# Autodesk Inventor assembly: MotorBlockModelisme
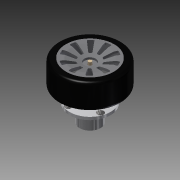
[picture p0: Inventor's stored thumbnail of the model, 180x180]
Saved by Autodesk Inventor 2014 SP1 (Build 180222100, 222)
## iProperties
Created: 2015-04-18
Part Number: MotorBlockModelisme
Document SubType Name: Assembly
Designer: david
Author: david
## Documents named in this file (5)
- C:\Users\asus\Documents\Autodesk\Projects\AUSBEEDone\Components\Motors\MotorBlockModelling.iam
- C:\Users\asus\Documents\Autodesk\Projects\AUSBEEDone\Components\Motors\Motor.iam
- C:\Users\asus\Documents\Autodesk\Projects\AUSBEEDone\Components\Modelling\Hub_Hex_12mm.ipt
- C:\Users\asus\Documents\Autodesk\Projects\AUSBEEDone\Components\Fasteners\Screw_CountersunkHead_3x10.ipt
- C:\Users\asus\Documents\Autodesk\Projects\AUSBEEDone\Components\Modelling\ModellingWheel_65mm.ipt
## Components (5 placed, 4 different names)
1. Motor:1 [sub-assembly] — Mate:1, Mate:2, Mate:5, Mate:6
2. ModellingWheel_65mm:1 — Mate:7, Angle:1, Mate:8
3. Hub_Hex_12mm:1 — Mate:1, Mate:2, Mate:3, Mate:4, Mate:7, Angle:1, Mate:8
4. Screw_CountersunkHead_3x10:1 — Mate:4, Mate:6
5. Screw_CountersunkHead_3x10:2 — Mate:3, Mate:5
## Relationships (9: Mate 8, Angle 1)
- Mate:1: Motor:1 ↔ Hub_Hex_12mm:1
- Mate:2: Motor:1 ↔ Hub_Hex_12mm:1
- Mate:3: Hub_Hex_12mm:1 ↔ Screw_CountersunkHead_3x10:2
- Mate:4: Hub_Hex_12mm:1 ↔ Screw_CountersunkHead_3x10:1
- Mate:5: Motor:1 ↔ Screw_CountersunkHead_3x10:2
- Mate:6: Motor:1 ↔ Screw_CountersunkHead_3x10:1
- Mate:7: ModellingWheel_65mm:1 ↔ Hub_Hex_12mm:1
- Angle:1 (180 deg): ModellingWheel_65mm:1 ↔ Hub_Hex_12mm:1
- Mate:8: ModellingWheel_65mm:1 ↔ Hub_Hex_12mm:1
